# Autodesk Inventor assembly: Conbadge2_Electro_Bugaloo
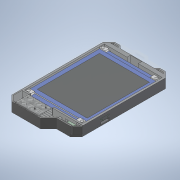
[picture p0: Inventor's stored thumbnail of the model, 180x180]
Saved by Autodesk Inventor 2020 (Build 240168000, 168)
## iProperties
Created: 2021-11-22
Part Number: Conbadge2_Electro_Bugaloo
Document SubType Name: Assembly
Designer: mtkts
Author: mtkts
## Documents named in this file (9)
- C:\Users\mtkts\AndroidStudioProjects\EPaperConbadge\Epaper-Conbadge-Github\3D Models\Conbadge2_Electro_Bugaloo.iam
- C:\Users\mtkts\AndroidStudioProjects\EPaperConbadge\Epaper-Conbadge-Github\3D Models\E-Paper Display.ipt
- C:\Users\mtkts\AndroidStudioProjects\EPaperConbadge\Epaper-Conbadge-Github\3D Models\Screen_Spacers.ipt
- C:\Users\mtkts\AndroidStudioProjects\EPaperConbadge\Epaper-Conbadge-Github\3D Models\Screen_Spacers_MIR.ipt
- C:\Users\mtkts\AndroidStudioProjects\EPaperConbadge\Epaper-Conbadge-Github\3D Models\Acrylic Panel.ipt
- C:\Users\mtkts\AndroidStudioProjects\EPaperConbadge\Epaper-Conbadge-Github\3D Models\Charger_Port.ipt
- C:\Users\mtkts\AndroidStudioProjects\EPaperConbadge\Epaper-Conbadge-Github\3D Models\Battery.ipt
- C:\Users\mtkts\AndroidStudioProjects\EPaperConbadge\Epaper-Conbadge-Github\3D Models\BMS.ipt
- C:\Users\mtkts\AndroidStudioProjects\EPaperConbadge\Epaper-Conbadge-Github\3D Models\Covering.ipt
## Components (10 placed, 8 different names)
1. E-Paper Display:1 — Flush:1, Mate:1, Flush:2, Mate:2, Mate:4, Mate:5, Flush:3, Flush:4, Mate:6, Mate:7, Angle:1, Mate:9, Mate:10, Mate:11, Angle:2, Flush:7
2. Screen_Spacers:1 — Flush:1, Flush:5
3. Screen_Spacers:2 — Flush:4, Mate:6, Mate:7
4. Screen_Spacers_MIR:1 — Mate:1, Flush:2, Mate:2
5. Screen_Spacers_MIR:2 — Mate:4, Mate:5, Flush:3
6. Acrylic Panel:1 — Flush:5, Mate:12, Flush:6
7. Charger_Port:1 — Mate:11, Angle:2
8. Battery:1 — Mate:12
9. BMS:1 — Angle:1, Mate:9, Mate:10
10. Covering:1 — Flush:6, Flush:7
## Relationships (19: Mate 10, Flush 7, Angle 2)
- Flush:1: E-Paper Display:1 ↔ Screen_Spacers:1
- Mate:1: E-Paper Display:1 ↔ Screen_Spacers_MIR:1
- Flush:2: E-Paper Display:1 ↔ Screen_Spacers_MIR:1
- Mate:2: E-Paper Display:1 ↔ Screen_Spacers_MIR:1
- Mate:4: E-Paper Display:1 ↔ Screen_Spacers_MIR:2
- Mate:5: E-Paper Display:1 ↔ Screen_Spacers_MIR:2
- Flush:3: E-Paper Display:1 ↔ Screen_Spacers_MIR:2
- Flush:4: E-Paper Display:1 ↔ Screen_Spacers:2
- Mate:6: E-Paper Display:1 ↔ Screen_Spacers:2
- Mate:7: E-Paper Display:1 ↔ Screen_Spacers:2
- Flush:5: Screen_Spacers:1 ↔ Acrylic Panel:1
- Angle:1 (0 deg): E-Paper Display:1 ↔ BMS:1
- Mate:9: E-Paper Display:1 ↔ BMS:1
- Mate:10: E-Paper Display:1 ↔ BMS:1
- Mate:11: E-Paper Display:1 ↔ Charger_Port:1
- Angle:2 (0 deg): E-Paper Display:1 ↔ Charger_Port:1
- Mate:12: Acrylic Panel:1 ↔ Battery:1
- Flush:6: Acrylic Panel:1 ↔ Covering:1
- Flush:7: E-Paper Display:1 ↔ Covering:1
